# Autodesk Inventor assembly: Toothed Belt 3M
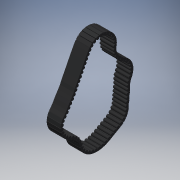
[picture p0: Inventor's stored thumbnail of the model, 180x180]
Saved by Autodesk Inventor 2019.2 (Build 232265000, 265)
## iProperties
Created: 2018-11-28
Part Number: Toothed Belt 3M
Document SubType Name: Assembly
Designer: Petar
Author: Petar
## Documents named in this file (2)
- D:\OMG\E-Board\CAD\Inventor\Mechanical Components\Toothed Belt 3M.iam
- D:\OMG\E-Board\CAD\Inventor\Mechanical Components\Toothed Belt Component.ipt
## Components (75 placed, 1 different names)
1. Toothed Belt Component:1 — Rotational:1, Rotational:75
2. Toothed Belt Component:2 — Rotational:1, Rotational:3
3. Toothed Belt Component:3 — Rotational:3
4. Toothed Belt Component:4 — Rotational:7
5. Toothed Belt Component:5 — Rotational:7
6. Toothed Belt Component:6
7. Toothed Belt Component:7
8. Toothed Belt Component:8 — Rotational:15
9. Toothed Belt Component:9 — Rotational:15
10. Toothed Belt Component:10
11. Toothed Belt Component:11
12. Toothed Belt Component:12
13. Toothed Belt Component:13
14. Toothed Belt Component:14
15. Toothed Belt Component:15
16. Toothed Belt Component:16 — Rotational:31
17. Toothed Belt Component:17 — Rotational:31
18. Toothed Belt Component:18
19. Toothed Belt Component:19
20. Toothed Belt Component:20
21. Toothed Belt Component:21
22. Toothed Belt Component:22
23. Toothed Belt Component:23
24. Toothed Belt Component:24
25. Toothed Belt Component:25
26. Toothed Belt Component:26
27. Toothed Belt Component:27
28. Toothed Belt Component:28
29. Toothed Belt Component:29
30. Toothed Belt Component:30
31. Toothed Belt Component:31
32. Toothed Belt Component:32 — Rotational:63
33. Toothed Belt Component:33 — Rotational:63
34. Toothed Belt Component:34
35. Toothed Belt Component:35
36. Toothed Belt Component:36
37. Toothed Belt Component:37
38. Toothed Belt Component:38
39. Toothed Belt Component:39
40. Toothed Belt Component:40
41. Toothed Belt Component:41
42. Toothed Belt Component:42
43. Toothed Belt Component:43
44. Toothed Belt Component:44
45. Toothed Belt Component:45
46. Toothed Belt Component:46
47. Toothed Belt Component:47
48. Toothed Belt Component:48
49. Toothed Belt Component:49
50. Toothed Belt Component:50
51. Toothed Belt Component:51
52. Toothed Belt Component:52
53. Toothed Belt Component:53
54. Toothed Belt Component:54
55. Toothed Belt Component:55
56. Toothed Belt Component:56
57. Toothed Belt Component:57
58. Toothed Belt Component:58
59. Toothed Belt Component:59
60. Toothed Belt Component:60
61. Toothed Belt Component:61
62. Toothed Belt Component:62
63. Toothed Belt Component:63
64. Toothed Belt Component:64 — Rotational:74
65. Toothed Belt Component:65 — Rotational:74
66. Toothed Belt Component:66
67. Toothed Belt Component:67
68. Toothed Belt Component:68
69. Toothed Belt Component:69
70. Toothed Belt Component:70
71. Toothed Belt Component:71
72. Toothed Belt Component:72
73. Toothed Belt Component:73
74. Toothed Belt Component:74
75. Toothed Belt Component:75 — Rotational:75
## Relationships (75: RevoluteJoint 75)
- Rotational:1 [RevoluteJoint]: Toothed Belt Component:1 ↔ Toothed Belt Component:2
- [RevoluteJoint]: Toothed Belt Component:3 ↔ Toothed Belt Component:4
- Rotational:3 [RevoluteJoint]: Toothed Belt Component:2 ↔ Toothed Belt Component:3
- [RevoluteJoint]: Toothed Belt Component:5 ↔ Toothed Belt Component:6
- [RevoluteJoint]: Toothed Belt Component:7 ↔ Toothed Belt Component:8
- [RevoluteJoint]: Toothed Belt Component:6 ↔ Toothed Belt Component:7
- Rotational:7 [RevoluteJoint]: Toothed Belt Component:4 ↔ Toothed Belt Component:5
- [RevoluteJoint]: Toothed Belt Component:9 ↔ Toothed Belt Component:10
- [RevoluteJoint]: Toothed Belt Component:11 ↔ Toothed Belt Component:12
- [RevoluteJoint]: Toothed Belt Component:10 ↔ Toothed Belt Component:11
- [RevoluteJoint]: Toothed Belt Component:13 ↔ Toothed Belt Component:14
- [RevoluteJoint]: Toothed Belt Component:15 ↔ Toothed Belt Component:16
- [RevoluteJoint]: Toothed Belt Component:14 ↔ Toothed Belt Component:15
- [RevoluteJoint]: Toothed Belt Component:12 ↔ Toothed Belt Component:13
- Rotational:15 [RevoluteJoint]: Toothed Belt Component:8 ↔ Toothed Belt Component:9
- [RevoluteJoint]: Toothed Belt Component:17 ↔ Toothed Belt Component:18
- [RevoluteJoint]: Toothed Belt Component:19 ↔ Toothed Belt Component:20
- [RevoluteJoint]: Toothed Belt Component:18 ↔ Toothed Belt Component:19
- [RevoluteJoint]: Toothed Belt Component:21 ↔ Toothed Belt Component:22
- [RevoluteJoint]: Toothed Belt Component:23 ↔ Toothed Belt Component:24
- [RevoluteJoint]: Toothed Belt Component:22 ↔ Toothed Belt Component:23
- [RevoluteJoint]: Toothed Belt Component:20 ↔ Toothed Belt Component:21
- [RevoluteJoint]: Toothed Belt Component:25 ↔ Toothed Belt Component:26
- [RevoluteJoint]: Toothed Belt Component:27 ↔ Toothed Belt Component:28
- [RevoluteJoint]: Toothed Belt Component:26 ↔ Toothed Belt Component:27
- [RevoluteJoint]: Toothed Belt Component:29 ↔ Toothed Belt Component:30
- [RevoluteJoint]: Toothed Belt Component:31 ↔ Toothed Belt Component:32
- [RevoluteJoint]: Toothed Belt Component:30 ↔ Toothed Belt Component:31
- [RevoluteJoint]: Toothed Belt Component:28 ↔ Toothed Belt Component:29
- [RevoluteJoint]: Toothed Belt Component:24 ↔ Toothed Belt Component:25
- Rotational:31 [RevoluteJoint]: Toothed Belt Component:16 ↔ Toothed Belt Component:17
- [RevoluteJoint]: Toothed Belt Component:33 ↔ Toothed Belt Component:34
- [RevoluteJoint]: Toothed Belt Component:35 ↔ Toothed Belt Component:36
- [RevoluteJoint]: Toothed Belt Component:34 ↔ Toothed Belt Component:35
- [RevoluteJoint]: Toothed Belt Component:37 ↔ Toothed Belt Component:38
- [RevoluteJoint]: Toothed Belt Component:39 ↔ Toothed Belt Component:40
- [RevoluteJoint]: Toothed Belt Component:38 ↔ Toothed Belt Component:39
- [RevoluteJoint]: Toothed Belt Component:36 ↔ Toothed Belt Component:37
- [RevoluteJoint]: Toothed Belt Component:41 ↔ Toothed Belt Component:42
- [RevoluteJoint]: Toothed Belt Component:43 ↔ Toothed Belt Component:44
- [RevoluteJoint]: Toothed Belt Component:42 ↔ Toothed Belt Component:43
- [RevoluteJoint]: Toothed Belt Component:45 ↔ Toothed Belt Component:46
- [RevoluteJoint]: Toothed Belt Component:47 ↔ Toothed Belt Component:48
- [RevoluteJoint]: Toothed Belt Component:46 ↔ Toothed Belt Component:47
- [RevoluteJoint]: Toothed Belt Component:44 ↔ Toothed Belt Component:45
- [RevoluteJoint]: Toothed Belt Component:40 ↔ Toothed Belt Component:41
- [RevoluteJoint]: Toothed Belt Component:49 ↔ Toothed Belt Component:50
- [RevoluteJoint]: Toothed Belt Component:51 ↔ Toothed Belt Component:52
- [RevoluteJoint]: Toothed Belt Component:50 ↔ Toothed Belt Component:51
- [RevoluteJoint]: Toothed Belt Component:53 ↔ Toothed Belt Component:54
- [RevoluteJoint]: Toothed Belt Component:55 ↔ Toothed Belt Component:56
- [RevoluteJoint]: Toothed Belt Component:54 ↔ Toothed Belt Component:55
- [RevoluteJoint]: Toothed Belt Component:52 ↔ Toothed Belt Component:53
- [RevoluteJoint]: Toothed Belt Component:57 ↔ Toothed Belt Component:58
- [RevoluteJoint]: Toothed Belt Component:59 ↔ Toothed Belt Component:60
- [RevoluteJoint]: Toothed Belt Component:58 ↔ Toothed Belt Component:59
- [RevoluteJoint]: Toothed Belt Component:61 ↔ Toothed Belt Component:62
- [RevoluteJoint]: Toothed Belt Component:63 ↔ Toothed Belt Component:64
- [RevoluteJoint]: Toothed Belt Component:62 ↔ Toothed Belt Component:63
- [RevoluteJoint]: Toothed Belt Component:60 ↔ Toothed Belt Component:61
- [RevoluteJoint]: Toothed Belt Component:56 ↔ Toothed Belt Component:57
- [RevoluteJoint]: Toothed Belt Component:48 ↔ Toothed Belt Component:49
- Rotational:63 [RevoluteJoint]: Toothed Belt Component:32 ↔ Toothed Belt Component:33
- [RevoluteJoint]: Toothed Belt Component:66 ↔ Toothed Belt Component:67
- [RevoluteJoint]: Toothed Belt Component:65 ↔ Toothed Belt Component:66
- [RevoluteJoint]: Toothed Belt Component:68 ↔ Toothed Belt Component:69
- [RevoluteJoint]: Toothed Belt Component:70 ↔ Toothed Belt Component:71
- [RevoluteJoint]: Toothed Belt Component:69 ↔ Toothed Belt Component:70
- [RevoluteJoint]: Toothed Belt Component:72 ↔ Toothed Belt Component:73
- [RevoluteJoint]: Toothed Belt Component:74 ↔ Toothed Belt Component:75
- [RevoluteJoint]: Toothed Belt Component:73 ↔ Toothed Belt Component:74
- [RevoluteJoint]: Toothed Belt Component:71 ↔ Toothed Belt Component:72
- [RevoluteJoint]: Toothed Belt Component:67 ↔ Toothed Belt Component:68
- Rotational:74 [RevoluteJoint]: Toothed Belt Component:64 ↔ Toothed Belt Component:65
- Rotational:75 [RevoluteJoint]: Toothed Belt Component:1 ↔ Toothed Belt Component:75
## Named parameters: d296_d0 = 0 mm, d297_d1 = 14.813453 deg, d298_d2 = 15 deg, d299_d3 = -15 deg, d304_d296_d0 = 0 mm, d305_d297_d1 = 14.784389 deg, d306_d298_d2 = 15 deg, d307_d299_d3 = -15 deg, d308_d300 = 0 mm, d309_d301 = 14.79303 deg, d310_d302 = 15 deg, d311_d303 = -15 deg, d312_d0 = 0 mm, d313_d1 = 14.79644 deg, d314_d2 = 15 deg, d315_d3 = -15 deg, d320_d304_d296_d0 = 0 mm, d321_d305_d297_d1 = 14.365844 deg, d322_d306_d298_d2 = 15 deg, d323_d307_d299_d3 = -15 deg, d324_d308_d300 = 0 mm, d325_d309_d301 = -14.697847 deg, d326_d310_d302 = 15 deg, d327_d311_d303 = -15 deg, d328_d312_d0 = 0 mm, d329_d313_d1 = -14.781251 deg, d330_d314_d2 = 15 deg, d331_d315_d3 = -15 deg, d332_d316 = 0 mm, d333_d317 = -14.844885 deg, d334_d318 = 15 deg, d335_d319 = -15 deg, d336_d296_d0 = 0 mm, d337_d297_d1 = -14.899481 deg, d338_d298_d2 = 15 deg, d339_d299_d3 = -15 deg, d340_d300 = 0 mm, d341_d301 = 2.030707 deg, d342_d302 = 15 deg, d343_d303 = -15 deg, d344_d0 = 0 mm, d345_d1 = -14.629417 deg, d346_d2 = 15 deg, d347_d3 = -15 deg, d352_d304_d296_d0 = 0 mm, d353_d305_d297_d1 = 14.999901 deg, d354_d306_d298_d2 = 15 deg, d355_d307_d299_d3 = -15 deg, d356_d308_d300 = 0 mm, d357_d309_d301 = 15 deg, d358_d310_d302 = 15 deg, d359_d311_d303 = -15 deg, d360_d312_d0 = 0 mm, d361_d313_d1 = 15 deg, d362_d314_d2 = 15 deg, d363_d315_d3 = -15 deg, d364_d316 = 0 mm, d365_d317 = 15 deg, d366_d318 = 15 deg, d367_d319 = -15 deg, d368_d320_d304_d296_d0 = 0 mm, d369_d321_d305_d297_d1 = -0.098502 deg, d370_d322_d306_d298_d2 = 15 deg, d371_d323_d307_d299_d3 = -15 deg, d372_d324_d308_d300 = 0 mm, d373_d325_d309_d301 = 0.072931 deg, d374_d326_d310_d302 = 15 deg, d375_d327_d311_d303 = -15 deg, d376_d328_d312_d0 = 0 mm, d377_d329_d313_d1 = 0.205933 deg, d378_d330_d314_d2 = 15 deg, d379_d331_d315_d3 = -15 deg, d380_d332_d316 = 0 mm, d381_d333_d317 = 0.312131 deg, d382_d334_d318 = 15 deg, d383_d335_d319 = -15 deg, d384_d336_d296_d0 = 0 mm, d385_d337_d297_d1 = 0.461879 deg, d386_d338_d298_d2 = 15 deg, d387_d339_d299_d3 = -15 deg, d388_d340_d300 = 0 mm, d389_d341_d301 = 3.093656 deg, d390_d342_d302 = 15 deg, d391_d343_d303 = -15 deg, d392_d344_d0 = 0 mm, d393_d345_d1 = 12.341044 deg, d394_d346_d2 = 15 deg, d395_d347_d3 = -15 deg, d396_d348 = 0 mm, d397_d349 = 14.999807 deg, d398_d350 = 15 deg, d399_d351 = -15 deg, d400_d296_d0 = 0 mm, d401_d297_d1 = 14.787137 deg, d402_d298_d2 = 15 deg, d403_d299_d3 = -15 deg, d404_d300 = 0 mm, d405_d301 = 14.341611 deg, d406_d302 = 15 deg, d407_d303 = -15 deg, d408_d0 = 0 mm, d409_d1 = 14.300011 deg, d410_d2 = 15 deg, d411_d3 = -15 deg, d416_d304_d296_d0 = 0 mm, d417_d305_d297_d1 = -4.832023 deg, d418_d306_d298_d2 = 15 deg, d419_d307_d299_d3 = -15 deg, d420_d308_d300 = 0 mm, d421_d309_d301 = 2.794107 deg, d422_d310_d302 = 15 deg, d423_d311_d303 = -15 deg, d424_d312_d0 = 0 mm, d425_d313_d1 = 1.593379 deg, d426_d314_d2 = 15 deg, d427_d315_d3 = -15 deg, d428_d316 = 0 mm, d429_d317 = -2.085427 deg, d430_d318 = 15 deg, d431_d319 = -15 deg, d432_d320_d304_d296_d0 = 0 mm, d433_d321_d305_d297_d1 = 14.297825 deg, d434_d322_d306_d298_d2 = 15 deg, d435_d323_d307_d299_d3 = -15 deg, d436_d324_d308_d300 = 0 mm, d437_d325_d309_d301 = 14.999999 deg, d438_d326_d310_d302 = 15 deg, d439_d327_d311_d303 = -15 deg, d440_d328_d312_d0 = 0 mm, d441_d329_d313_d1 = 14.577953 deg, d442_d330_d314_d2 = 15 deg, d443_d331_d315_d3 = -15 deg, d444_d332_d316 = 0 mm, d445_d333_d317 = 14.901987 deg, d446_d334_d318 = 15 deg, d447_d335_d319 = -15 deg, d448_d336_d296_d0 = 0 mm, d449_d337_d297_d1 = 15 deg, d450_d338_d298_d2 = 15 deg, d451_d339_d299_d3 = -15 deg, d452_d340_d300 = 0 mm, d453_d341_d301 = 14.999946 deg, d454_d342_d302 = 15 deg, d455_d343_d303 = -15 deg, d456_d344_d0 = 0 mm, d457_d345_d1 = 14.999976 deg, d458_d346_d2 = 15 deg, d459_d347_d3 = -15 deg, d460_d348 = 0 mm, d461_d349 = -5.549044 deg, d462_d350 = 15 deg, d463_d351 = -15 deg, d464_d412 = 0 mm, d465_d413 = 2.014825 deg, d466_d414 = 15 deg, d467_d415 = -15 deg, d468_d352_d304_d296_d0 = 0 mm, d469_d353_d305_d297_d1 = 13.662888 deg, d470_d354_d306_d298_d2 = 15 deg, d471_d355_d307_d299_d3 = -15 deg, d472_d356_d308_d300 = 0 mm, d473_d357_d309_d301 = 14.255087 deg, d474_d358_d310_d302 = 15 deg, d475_d359_d311_d303 = -15 deg, d476_d360_d312_d0 = 0 mm, d477_d361_d313_d1 = 11.880164 deg, d478_d362_d314_d2 = 15 deg, d479_d363_d315_d3 = -15 deg, d480_d364_d316 = 0 mm, d481_d365_d317 = -13.284976 deg, d482_d366_d318 = 15 deg, d483_d367_d319 = -15 deg, d484_d368_d320_d304_d296_d0 = 0 mm, d485_d369_d321_d305_d297_d1 = -0.357201 deg, d486_d370_d322_d306_d298_d2 = 15 deg, d487_d371_d323_d307_d299_d3 = -15 deg, d488_d372_d324_d308_d300 = 0 mm, d489_d373_d325_d309_d301 = 6.518512 deg, d490_d374_d326_d310_d302 = 15 deg, d491_d375_d327_d311_d303 = -15 deg, d492_d376_d328_d312_d0 = 0 mm, d493_d377_d329_d313_d1 = 7.603314 deg, d494_d378_d330_d314_d2 = 15 deg, d495_d379_d331_d315_d3 = -15 deg, d496_d380_d332_d316 = 0 mm, d497_d381_d333_d317 = 8.725572 deg, d498_d382_d334_d318 = 15 deg, d499_d383_d335_d319 = -15 deg, d500_d384_d336_d296_d0 = 0 mm, d501_d385_d337_d297_d1 = 9.848586 deg, d502_d386_d338_d298_d2 = 15 deg, d503_d387_d339_d299_d3 = -15 deg, d504_d388_d340_d300 = 0 mm, d505_d389_d341_d301 = 10.943313 deg, d506_d390_d342_d302 = 15 deg, d507_d391_d343_d303 = -15 deg, d508_d392_d344_d0 = 0 mm, d509_d393_d345_d1 = 11.972173 deg, d510_d394_d346_d2 = 15 deg, d511_d395_d347_d3 = -15 deg, d512_d396_d348 = 0 mm, d513_d397_d349 = 12.892203 deg, d514_d398_d350 = 15 deg, d515_d399_d351 = -15 deg, d516_d400_d296_d0 = 0 mm, d517_d401_d297_d1 = -11.517438 deg, d518_d402_d298_d2 = 15 deg, d519_d403_d299_d3 = -15 deg, d520_d404_d300 = 0 mm, d521_d405_d301 = -15 deg, d522_d406_d302 = 15 deg, d523_d407_d303 = -15 deg, d524_d408_d0 = 0 mm, d525_d409_d1 = -15 deg, d526_d410_d2 = 15 deg, d527_d411_d3 = -15 deg, d528_d296_d0 = 0 mm, d529_d297_d1 = -9.20722 deg, d530_d298_d2 = 15 deg, d531_d299_d3 = -15 deg, d532_d300 = 0 mm, d533_d301 = 5.577088 deg, d534_d302 = 15 deg, d535_d303 = -15 deg, d536_d0 = 0 mm, d537_d1 = -0.443509 deg, d538_d2 = 15 deg, d539_d3 = -15 deg, d544_d508_d392_d344_d0 = 0 mm, d545_d509_d393_d345_d1 = 15 deg, d546_d510_d394_d346_d2 = 15 deg, d547_d511_d395_d347_d3 = -15 deg, d548_d512_d396_d348 = 0 mm, d549_d513_d397_d349 = 15 deg, d550_d514_d398_d350 = 15 deg, d551_d515_d399_d351 = -15 deg, d552_d468_d352_d304_d296_d0 = 0 mm, d553_d469_d353_d305_d297_d1 = 5.904992 deg, d554_d470_d354_d306_d298_d2 = 15 deg, d555_d471_d355_d307_d299_d3 = -15 deg, d556_d472_d356_d308_d300 = 0 mm, d557_d473_d357_d309_d301 = -0.577596 deg, d558_d474_d358_d310_d302 = 15 deg, d559_d475_d359_d311_d303 = -15 deg, d560_d484_d368_d320_d304_d296_d0 = 0 mm, d561_d485_d369_d321_d305_d297_d1 = 13.016961 deg, d562_d486_d370_d322_d306_d298_d2 = 15 deg, d563_d487_d371_d323_d307_d299_d3 = -15 deg, d564_d488_d372_d324_d308_d300 = 0 mm, d565_d489_d373_d325_d309_d301 = -14.908353 deg, d566_d490_d374_d326_d310_d302 = 15 deg, d567_d491_d375_d327_d311_d303 = -15 deg, d568_d492_d376_d328_d312_d0 = 0 mm, d569_d493_d377_d329_d313_d1 = 14.81785 deg, d570_d494_d378_d330_d314_d2 = 15 deg, d571_d495_d379_d331_d315_d3 = -15 deg, d572_d496_d380_d332_d316 = 0 mm, d573_d497_d381_d333_d317 = -14.999999 deg, d574_d498_d382_d334_d318 = 15 deg, d575_d499_d383_d335_d319 = -15 deg, d576_d500_d384_d336_d296_d0 = 0 mm, d577_d501_d385_d337_d297_d1 = 14.999988 deg, d578_d502_d386_d338_d298_d2 = 15 deg, d579_d503_d387_d339_d299_d3 = -15 deg, d580_d504_d388_d340_d300 = 0 mm, d581_d505_d389_d341_d301 = 12.422228 deg, d582_d506_d390_d342_d302 = 15 deg, d583_d507_d391_d343_d303 = -15 deg
